# Autodesk Inventor assembly: Ensemble - Glissiere Gauche
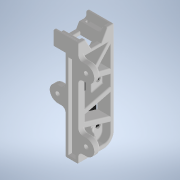
[picture p0: Inventor's stored thumbnail of the model, 180x180]
Saved by Autodesk Inventor 2021 (Build 250183000, 183)
## iProperties
Created: 2021-01-25
Part Number: Ensemble - Glissiere Gauche
Document SubType Name: Assembly
Designer: dimercur
Author: dimercur
## Documents named in this file (4)
- C:\Users\dimercur\Travail\Projets Git\voilier\meca\Equerres porte carte\Ensemble - Glissiere Gauche.iam
- C:\Users\dimercur\Travail\Projets Git\voilier\meca\Equerres porte carte\Fixation gauche.ipt
- C:\Users\dimercur\Travail\Projets Git\voilier\meca\Equerres porte carte\RDC-250.ipt
- RDC-250.ipt
## Components (2 placed, 2 different names)
1. Fixation Gauche:1 — Placage:1, Placage:2, Placage:3
2. RDC-250:1 — Placage:1, Placage:2, Placage:3
## Relationships (3: Mate 3)
- Placage:1 [Mate]: Fixation Gauche:1 ↔ RDC-250:1
- Placage:2 [Mate]: Fixation Gauche:1 ↔ RDC-250:1
- Placage:3 [Mate]: Fixation Gauche:1 ↔ RDC-250:1
